# Autodesk Inventor assembly: Stress Test Assem
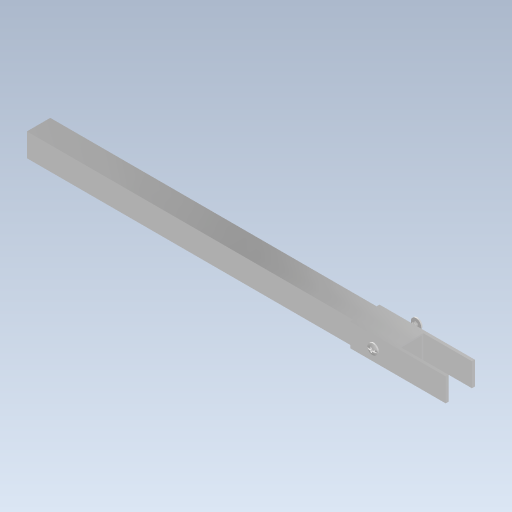
[picture p0: Inventor's stored thumbnail of the model, 512x512]
Saved by Autodesk Inventor 2023 (Build 270158000, 158)
## iProperties
Created: 2023-03-23
Part Number: Stress Test Assem
Document SubType Name: Assembly
Designer: Dave
Author: Dave
## Documents named in this file (5)
- C:\Users\Dave\Documents\GitHub\BehrendURCMechanical\CAD\Chassis V3\Pivot Stress Test\Stress Test Assem.iam
- C:\Users\Dave\Downloads\98002A207_Steel Binding Barrels and Screws.ipt
- C:\Users\Dave\Documents\GitHub\BehrendURCMechanical\CAD\Chassis V3\Pivot Stress Test\Channel\Part1-01.ipt
- C:\Users\Dave\Documents\GitHub\BehrendURCMechanical\CAD\Chassis V3\Pivot Stress Test\Channel.ipt
- C:\Users\Dave\Documents\GitHub\BehrendURCMechanical\CAD\Chassis V3\Pivot Stress Test\Plate.ipt
## Components (4 placed, 3 different names)
1. 98002A207_Steel Binding Barrels and Screws:1 — Insert:1
2. Part1-01:1 — Mate:1, Mate:2, Mate:3, Mate:4, Flush:1, Flush:2
3. Plate:1 — Mate:1, Mate:3, Flush:1, Insert:1
4. Plate:2 — Mate:2, Mate:4, Flush:2
## Relationships (7: Mate 4, Flush 2, Insert 1)
- Mate:1: Part1-01:1 ↔ Plate:1
- Mate:2: Part1-01:1 ↔ Plate:2
- Mate:3: Part1-01:1 ↔ Plate:1
- Mate:4: Part1-01:1 ↔ Plate:2
- Flush:1: Part1-01:1 ↔ Plate:1
- Flush:2: Part1-01:1 ↔ Plate:2
- Insert:1: 98002A207_Steel Binding Barrels and Screws:1 ↔ Plate:1
